# Autodesk Inventor assembly: Rocket Assemly
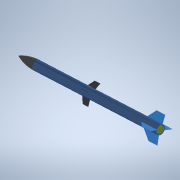
[picture p0: Inventor's stored thumbnail of the model, 180x180]
Saved by Autodesk Inventor 2020 (Build 240168000, 168)
## iProperties
Created: 2022-11-08
Part Number: Rocket Assemly
Document SubType Name: Assembly
Designer: Hp
Author: Hp
## Documents named in this file (14)
- E:\School\MechT 5.2\Project\Rocket\Rocket Assemly.iam
- E:\School\MechT 5.2\Project\Rocket\Body Tube.ipt
- E:\School\MechT 5.2\Project\Rocket\Nose.ipt
- E:\School\MechT 5.2\Project\Rocket\Tail Fin.ipt
- E:\School\MechT 5.2\Project\Rocket\Canard Fin.ipt
- E:\School\MechT 5.2\Project\Rocket\Launch lug.ipt
- E:\School\MechT 5.2\Project\Rocket\Parachute.ipt
- E:\School\MechT 5.2\Project\Rocket\ESP Cam.ipt
- E:\School\MechT 5.2\Project\Rocket\Flight Computer.ipt
- E:\School\MechT 5.2\Project\Rocket\Ejection Chamber.ipt
- E:\School\MechT 5.2\Project\Rocket\Mass.ipt
- E:\School\MechT 5.2\Project\Rocket\Engine.ipt
- E:\School\MechT 5.2\Project\Rocket\Shock cord.ipt
- E:\School\MechT 5.2\Project\Rocket\Battery.ipt
## Components (19 placed, 13 different names)
1. Body Tube:1 — Mate:1, Mate:2, Tangent:1, Angle:1, Tangent:2, Tangent:3, Mate:3, Tangent:4, Flush:1, Mate:4, Mate:5, Mate:9, Flush:3, Mate:10, Flush:4, Mate:11, Flush:5, Mate:12, Flush:6, Mate:13, Flush:7, Flush:8, Mate:14, Flush:9, Mate:15
2. Nose:1 — Mate:1, Mate:2, Mate:6, Mate:7
3. Launch lug:1 — Tangent:4, Flush:1
4. Parachute:1 — Mate:6, Mate:7
5. ESP Cam:1 — Mate:9, Flush:3
6. Flight Computer:1 — Mate:10, Flush:4
7. Ejection Chamber:1 — Mate:11, Flush:5
8. Mass:1 — Mate:12, Flush:6
9. Engine:1 — Mate:13, Flush:7
10. Shock cord:1 — Flush:8, Mate:14
11. Battery:1 — Flush:9, Mate:15
12. Tail Fin:3 — Tangent:1, Angle:1, Tangent:2, Mate:5
13. Tail Fin:4
14. Tail Fin:5
15. Tail Fin:6
16. Canard Fin:1 — Tangent:3, Mate:3
17. Canard Fin:2
18. Canard Fin:3 — Mate:4
19. Canard Fin:4
## Component patterns: (4 elements, first: Tail Fin:3), (4 elements, first: Canard Fin:1)
## Relationships (27: Mate 14, Flush 8, Tangent 4, Angle 1)
- Mate:1: Body Tube:1 ↔ Nose:1
- Mate:2: Body Tube:1 ↔ Nose:1
- Tangent:1: Body Tube:1 ↔ Tail Fin:3
- Angle:1 (90 deg): Body Tube:1 ↔ Tail Fin:3
- Tangent:2: Body Tube:1 ↔ Tail Fin:3
- Tangent:3: Body Tube:1 ↔ Canard Fin:1
- Mate:3 (39.5 mm): Body Tube:1 ↔ Canard Fin:1
- Tangent:4: Body Tube:1 ↔ Launch lug:1
- Flush:1 (-730 mm): Body Tube:1 ↔ Launch lug:1
- Mate:4 (-450 mm): Body Tube:1 ↔ Canard Fin:3
- Mate:5: Body Tube:1 ↔ Tail Fin:3
- Mate:6: Nose:1 ↔ Parachute:1
- Mate:7: Nose:1 ↔ Parachute:1
- Mate:9: Body Tube:1 ↔ ESP Cam:1
- Flush:3 (515 mm): Body Tube:1 ↔ ESP Cam:1
- Mate:10: Body Tube:1 ↔ Flight Computer:1
- Flush:4 (585 mm): Body Tube:1 ↔ Flight Computer:1
- Mate:11: Body Tube:1 ↔ Ejection Chamber:1
- Flush:5 (665 mm): Body Tube:1 ↔ Ejection Chamber:1
- Mate:12: Body Tube:1 ↔ Mass:1
- Flush:6 (795 mm): Body Tube:1 ↔ Mass:1
- Mate:13: Body Tube:1 ↔ Engine:1
- Flush:7: Body Tube:1 ↔ Engine:1
- Flush:8 (910 mm): Body Tube:1 ↔ Shock cord:1
- Mate:14: Body Tube:1 ↔ Shock cord:1
- Flush:9 (350 mm): Body Tube:1 ↔ Battery:1
- Mate:15: Body Tube:1 ↔ Battery:1
